# Autodesk Inventor assembly: speaker_assembly_v2
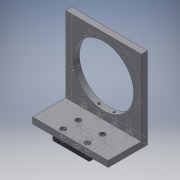
[picture p0: Inventor's stored thumbnail of the model, 180x180]
Saved by Autodesk Inventor 2019 (Build 230136000, 136)
## iProperties
Created: 2019-03-08
Part Number: speaker_assembly_v2
Document SubType Name: Assembly
Designer: Wilson Lab
Author: Wilson Lab
## Documents named in this file (4)
- C:\code\auditory-behavior-experiments\design-files\speaker-mount\speaker_assembly_v2.iam
- C:\code\auditory-behavior-experiments\design-files\speaker-mount\face_part.ipt
- C:\code\auditory-behavior-experiments\design-files\speaker-mount\base_part.ipt
- C:\code\auditory-behavior-experiments\design-files\speaker-mount\BA2-Solidworks.ipt
## Components (3 placed, 3 different names)
1. face_part:1 — Flush:1, Mate:1, Flush:2
2. base_part:1 — Flush:1, Mate:1, Flush:2
3. BA2-Solidworks:1
## Relationships (3: Flush 2, Mate 1)
- Flush:1: face_part:1 ↔ base_part:1
- Mate:1: face_part:1 ↔ base_part:1
- Flush:2: face_part:1 ↔ base_part:1
